# Autodesk Inventor assembly: Assembly1
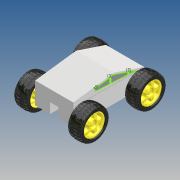
[picture p0: Inventor's stored thumbnail of the model, 180x180]
Saved by Autodesk Inventor 2020 (Build 240168000, 168)
## iProperties
Created: 2019-12-06
Part Number: Assembly1
Document SubType Name: Assembly
Designer: Berkant
Author: Berkant
## Documents named in this file (4)
- C:\Users\berka\Desktop\School\Project 2\Prototype 2\Assembly1.iam
- C:\Users\berka\Desktop\School\Project 2\Prototype 2\prototype 2.ipt
- C:\Users\berka\Desktop\Arduino Gear Motor.ipt
- C:\Users\berka\Desktop\wheel (scaled).ipt
## Components (9 placed, 3 different names)
1. prototype 2:1 — Rigid:1, Rigid:2, Rigid:3, Rigid:4
2. Arduino Gear Motor:1 — Rigid:1, Rotational:1
3. Arduino Gear Motor:2 — Rigid:2, Rotational:2
4. Arduino Gear Motor:3 — Rigid:4, Rotational:4
5. Arduino Gear Motor:4 — Rigid:3, Rotational:3
6. wheel (scaled):1 — Rotational:2
7. wheel (scaled):2 — Rotational:1
8. wheel (scaled):3 — Rotational:3
9. wheel (scaled):4 — Rotational:4
## Relationships (8: WeldJoint 4, RevoluteJoint 4)
- Rigid:1 [WeldJoint]: prototype 2:1 ↔ Arduino Gear Motor:1
- Rigid:2 [WeldJoint]: prototype 2:1 ↔ Arduino Gear Motor:2
- Rigid:3 [WeldJoint]: prototype 2:1 ↔ Arduino Gear Motor:4
- Rigid:4 [WeldJoint]: prototype 2:1 ↔ Arduino Gear Motor:3
- Rotational:1 [RevoluteJoint] (8.89 mm): Arduino Gear Motor:1 ↔ wheel (scaled):2
- Rotational:2 [RevoluteJoint] (8.636 mm): Arduino Gear Motor:2 ↔ wheel (scaled):1
- Rotational:3 [RevoluteJoint] (8.89 mm): Arduino Gear Motor:4 ↔ wheel (scaled):3
- Rotational:4 [RevoluteJoint] (8.89 mm): Arduino Gear Motor:3 ↔ wheel (scaled):4
